# Autodesk Inventor assembly: PlanetaryGear2
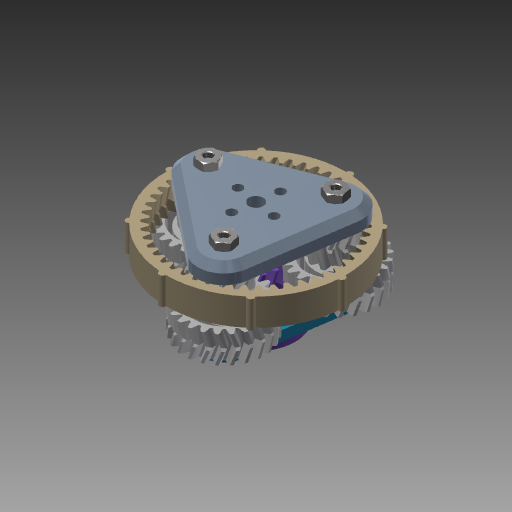
[picture p0: Inventor's stored thumbnail of the model, 512x512]
Saved by Autodesk Inventor 2019.1 (Build 231200000, 200)
## iProperties
Created: 2019-01-01
Part Number: PlanetaryGear2
Material: Generisch
Document SubType Name: Assembly
Designer: JochenAlt
Author: JochenAlt
## Documents named in this file (10)
- D:\Projects\Ondine\CAD\PlanetaryGear2\PlanetaryGearConstruction\PlanetaryGear2.iam
- D:\Projects\Ondine\CAD\PlanetaryGear2\PlanetaryGearConstruction\Stirnzahnrad21.ipt
- D:\Projects\Ondine\CAD\PlanetaryGear2\PlanetaryGearConstruction\PlanetaryWheel.iam
- D:\Projects\Ondine\CAD\PlanetaryGear2\PlanetaryGearConstruction\Top.ipt
- D:\Projects\Ondine\CAD\Bearings\W 627_7-2ZS.iam
- D:\Projects\Ondine\CAD\PlanetaryGear2\PlanetaryGearConstruction\Stirnzahnrad2-21.ipt
- D:\Projects\Ondine\CAD\PlanetaryGear2\PlanetaryGearConstruction\Bottom.ipt
- D:\Projects\Ondine\CAD\Mounting Hub 4mm.ipt
- C:\Users\JochenAlt\Documents\Inventor\Content Center Files\R2019\de-DE\BS 3692(1)\BS 3692 - M3(1).ipt
- C:\Users\JochenAlt\Documents\Inventor\Content Center Files\R2019\de-DE\DIN 912\DIN 912 - M3 x 0,5 x 25 x 18.ipt
## Components (21 placed, 9 different names)
1. Stirnzahnrad2:1 — Fluchtend:2, Fluchtend:3, Fluchtend:4, Passend:45
2. PlanetaryWheel:1 [sub-assembly] — Passend:10, Passend:17, Passend:20, Drehung:2, Passend:32, Fluchtend:2
3. PlanetaryWheel:2 [sub-assembly] — Passend:11, Passend:12, Passend:19, Passend:21, Drehung:3, Passend:35, Fluchtend:3, Fluchtend:5
4. PlanetaryWheel:3 [sub-assembly] — Passend:13, Passend:18, Passend:22, Passend:36, Fluchtend:4
5. W 627_7-2ZS:1 [sub-assembly] — Passend:10, Passend:31, Passend:32
6. W 627_7-2ZS:2 [sub-assembly] — Passend:11, Passend:12, Passend:33, Passend:35, Passend:40
7. W 627_7-2ZS:3 [sub-assembly] — Passend:13, Passend:34, Passend:36
8. Sun:2 — Passend:26, Passend:27, Passend:28, Drehung:1, Drehung:2, Drehung:3, Passend:44, Passend:45, Fluchtend:5
9. W 627_7-2ZS:4 [sub-assembly] — Passend:17, Passend:20, Passend:37
10. W 627_7-2ZS:5 [sub-assembly] — Passend:18, Passend:22, Passend:25
11. W 627_7-2ZS:6 [sub-assembly] — Passend:19, Passend:21, Passend:38
12. Bottom:1 — Passend:25, Drehung:1, Passend:37, Passend:38, Passend:44, Passend:46, Passend:48, Passend:50, Passend:58, Passend:59, Passend:60
13. Mounting Hub 4mm:1 — Passend:26, Passend:27, Passend:28
14. Top:1 — Passend:31, Passend:33, Passend:34, Passend:40, Passend:42, Passend:43, Passend:53, Passend:55, Passend:57
15. Mounting Hub 4mm:2 — Passend:42, Passend:43
16. DIN 912 - ersetzt durch DIN EN ISO 4762 M3 x 25:1 — Passend:46, Passend:52, Passend:58
17. DIN 912 - ersetzt durch DIN EN ISO 4762 M3 x 25:2 — Passend:48, Passend:56, Passend:60
18. DIN 912 - ersetzt durch DIN EN ISO 4762 M3 x 25:3 — Passend:50, Passend:54, Passend:59
19. BS 3692 - Metrisch M3:1 — Passend:52, Passend:53
20. BS 3692 - Metrisch M3:2 — Passend:54, Passend:55
21. BS 3692 - Metrisch M3:3 — Passend:56, Passend:57
## Relationships (46: Mate 39, Flush 4, RelateRotation 3)
- Passend:10 [Mate]: PlanetaryWheel:1 ↔ W 627_7-2ZS:1
- Passend:11 [Mate]: PlanetaryWheel:2 ↔ W 627_7-2ZS:2
- Passend:12 [Mate]: PlanetaryWheel:2 ↔ W 627_7-2ZS:2
- Passend:13 [Mate]: PlanetaryWheel:3 ↔ W 627_7-2ZS:3
- Passend:17 [Mate]: PlanetaryWheel:1 ↔ W 627_7-2ZS:4
- Passend:18 [Mate]: PlanetaryWheel:3 ↔ W 627_7-2ZS:5
- Passend:19 [Mate]: PlanetaryWheel:2 ↔ W 627_7-2ZS:6
- Passend:20 [Mate]: PlanetaryWheel:1 ↔ W 627_7-2ZS:4
- Passend:21 [Mate]: PlanetaryWheel:2 ↔ W 627_7-2ZS:6
- Passend:22 [Mate]: PlanetaryWheel:3 ↔ W 627_7-2ZS:5
- Passend:25 [Mate]: W 627_7-2ZS:5 ↔ Bottom:1
- Passend:26 [Mate]: Sun:2 ↔ Mounting Hub 4mm:1
- Passend:27 [Mate]: Sun:2 ↔ Mounting Hub 4mm:1
- Passend:28 [Mate]: Sun:2 ↔ Mounting Hub 4mm:1
- Drehung:1 [RelateRotation] (0.1111 ul): Sun:2 ↔ Bottom:1
- Drehung:2 [RelateRotation] (3 ul): PlanetaryWheel:1 ↔ Sun:2
- Drehung:3 [RelateRotation] (3 ul): PlanetaryWheel:2 ↔ Sun:2
- Passend:31 [Mate]: W 627_7-2ZS:1 ↔ Top:1
- Passend:32 [Mate]: PlanetaryWheel:1 ↔ W 627_7-2ZS:1
- Passend:33 [Mate]: W 627_7-2ZS:2 ↔ Top:1
- Passend:34 [Mate]: W 627_7-2ZS:3 ↔ Top:1
- Passend:35 [Mate]: PlanetaryWheel:2 ↔ W 627_7-2ZS:2
- Passend:36 [Mate]: PlanetaryWheel:3 ↔ W 627_7-2ZS:3
- Passend:37 [Mate]: W 627_7-2ZS:4 ↔ Bottom:1
- Passend:38 [Mate]: W 627_7-2ZS:6 ↔ Bottom:1
- Fluchtend:2 [Flush]: Stirnzahnrad2:1 ↔ PlanetaryWheel:1
- Fluchtend:3 [Flush]: Stirnzahnrad2:1 ↔ PlanetaryWheel:2
- Fluchtend:4 [Flush]: Stirnzahnrad2:1 ↔ PlanetaryWheel:3
- Passend:40 [Mate]: W 627_7-2ZS:2 ↔ Top:1
- Passend:42 [Mate]: Top:1 ↔ Mounting Hub 4mm:2
- Passend:43 [Mate]: Top:1 ↔ Mounting Hub 4mm:2
- Passend:44 [Mate]: Sun:2 ↔ Bottom:1
- Passend:45 [Mate]: Stirnzahnrad2:1 ↔ Sun:2
- Fluchtend:5 [Flush]: PlanetaryWheel:2 ↔ Sun:2
- Passend:46 [Mate]: Bottom:1 ↔ DIN 912 - ersetzt durch DIN EN ISO 4762 M3 x 25:1
- Passend:48 [Mate]: Bottom:1 ↔ DIN 912 - ersetzt durch DIN EN ISO 4762 M3 x 25:2
- Passend:50 [Mate]: Bottom:1 ↔ DIN 912 - ersetzt durch DIN EN ISO 4762 M3 x 25:3
- Passend:52 [Mate]: DIN 912 - ersetzt durch DIN EN ISO 4762 M3 x 25:1 ↔ BS 3692 - Metrisch M3:1
- Passend:53 [Mate]: Top:1 ↔ BS 3692 - Metrisch M3:1
- Passend:54 [Mate]: DIN 912 - ersetzt durch DIN EN ISO 4762 M3 x 25:3 ↔ BS 3692 - Metrisch M3:2
- Passend:55 [Mate]: Top:1 ↔ BS 3692 - Metrisch M3:2
- Passend:56 [Mate]: DIN 912 - ersetzt durch DIN EN ISO 4762 M3 x 25:2 ↔ BS 3692 - Metrisch M3:3
- Passend:57 [Mate]: Top:1 ↔ BS 3692 - Metrisch M3:3
- Passend:58 [Mate]: Bottom:1 ↔ DIN 912 - ersetzt durch DIN EN ISO 4762 M3 x 25:1
- Passend:59 [Mate]: Bottom:1 ↔ DIN 912 - ersetzt durch DIN EN ISO 4762 M3 x 25:3
- Passend:60 [Mate]: Bottom:1 ↔ DIN 912 - ersetzt durch DIN EN ISO 4762 M3 x 25:2
